# Autodesk Inventor assembly: MG-LT24
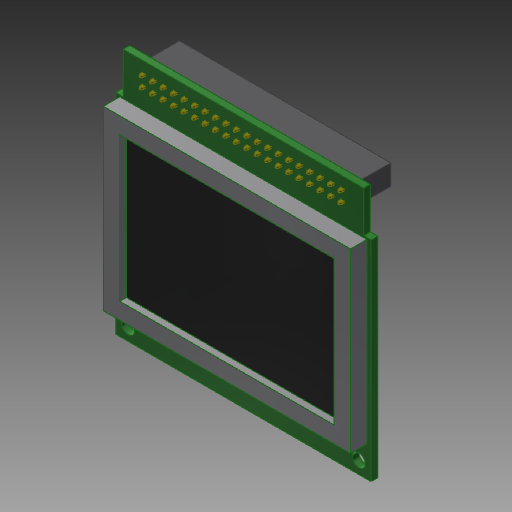
[picture p0: Inventor's stored thumbnail of the model, 512x512]
Saved by Autodesk Inventor 2019.4 (Build 234330000, 330)
## iProperties
Created: 2015-08-09
Part Number: MG-LT24
Document SubType Name: Assembly
Designer: rYan
Mass: 20.3599 g
Surface Area: 121.524 cm^2
Volume: 15.2846 cm^3
Density: 1.33205 g/cm^3
Author: rYan
## Documents named in this file (3)
- D:\TIGERsGIT\Hardware\mechanik\2020\Inventor\Purchased Parts\MG-LT24.iam
- D:\TIGERsGIT\Hardware\mechanik\2020\Inventor\Purchased Parts\LT24.ipt
- D:\TIGERsGIT\Hardware\mechanik\2020\Inventor\Purchased Parts\SSW-120-01-F-D\SSW-120-01-F-D.iam
## Components (2 placed, 2 different names)
1. LT24:1 — Passend:1, Fluchtend:1, Fluchtend:2
2. SSW-120-01-F-D:1 [sub-assembly] — Passend:1, Fluchtend:1, Fluchtend:2
## Relationships (3: Flush 2, Mate 1)
- Passend:1 [Mate]: LT24:1 ↔ SSW-120-01-F-D:1
- Fluchtend:1 [Flush]: LT24:1 ↔ SSW-120-01-F-D:1
- Fluchtend:2 [Flush] (1.5 mm): LT24:1 ↔ SSW-120-01-F-D:1
